# Autodesk Inventor assembly: Сборка1
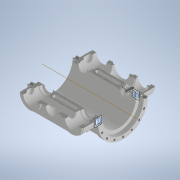
[picture p0: Inventor's stored thumbnail of the model, 180x180]
Saved by Autodesk Inventor 2021 (Build 250183000, 183)
## iProperties
Created: 2020-11-15
Part Number: Сборка1
Document SubType Name: Assembly
Designer: Тимоха
Author: Тимоха
## Documents named in this file (7)
- C:\Users\Тимоха\Desktop\КР Компрессор\МОЕ\Сборка1.iam
- C:\Users\Тимоха\Desktop\КР Компрессор\МОЕ\Цилиндр2.ipt
- C:\Users\Тимоха\Desktop\КР Компрессор\МОЕ\Прокладка рубашки охлаждения.ipt
- C:\Users\Тимоха\Desktop\КР Компрессор\МОЕ\Крышка рубашки охлаждения.ipt
- C:\Users\Тимоха\Documents\Inventor\Content Center Files\R2021\ru-RU\Bolt GOST R 50274-92\Болт M8-6g×20-F ГОСТ Р 50274-92.ipt
- C:\Users\Тимоха\Desktop\КР Компрессор\МОЕ\Клапан2.iam
- C:\Users\Тимоха\Desktop\КР Компрессор\МОЕ\Стакан1.ipt
## Components (7 placed, 6 different names)
1. Цилиндр2:1 — Заподлицо:1, Заподлицо:2, Жесткий:1, Жесткий:2, Жесткий:3, С поворотом:1
2. Прокладка рубашки охлаждения:1 — Заподлицо:2, Заподлицо:3, Жесткий:2, Заподлицо:4, Заподлицо:5
3. Прокладка рубашки охлаждения:2 — Жесткий:1
4. Крышка рубашки охлаждения:1 — Заподлицо:4, Заподлицо:5
5. Болт ГОСТ Р 50274-92 M8-6g×20-F:1 — Жесткий:3
6. Клапан2:1 [sub-assembly] — С поворотом:1, Жесткий:4
7. Стакан1:1 — Жесткий:4
## Relationships (10: Flush 5, WeldJoint 4, RevoluteJoint 1)
- Заподлицо:1 [Flush] (150.75 mm): Цилиндр2:1
- Заподлицо:2 [Flush]: Цилиндр2:1 ↔ Прокладка рубашки охлаждения:1
- Заподлицо:3 [Flush]: Прокладка рубашки охлаждения:1
- Жесткий:1 [WeldJoint]: Цилиндр2:1 ↔ Прокладка рубашки охлаждения:2
- Жесткий:2 [WeldJoint]: Цилиндр2:1 ↔ Прокладка рубашки охлаждения:1
- Заподлицо:4 [Flush]: Прокладка рубашки охлаждения:1 ↔ Крышка рубашки охлаждения:1
- Заподлицо:5 [Flush]: Прокладка рубашки охлаждения:1 ↔ Крышка рубашки охлаждения:1
- Жесткий:3 [WeldJoint] (5 mm): Цилиндр2:1 ↔ Болт ГОСТ Р 50274-92 M8-6g×20-F:1
- С поворотом:1 [RevoluteJoint]: Цилиндр2:1 ↔ Клапан2:1
- Жесткий:4 [WeldJoint]: Клапан2:1 ↔ Стакан1:1
